# Autodesk Inventor assembly: ASY PNS-002 right module
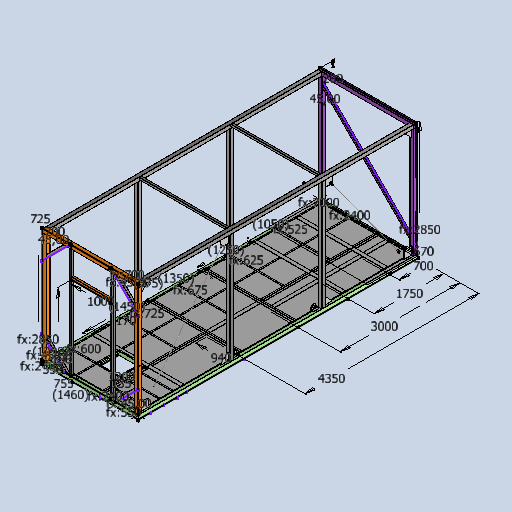
[picture p0: Inventor's stored thumbnail of the model, 512x512]
Saved by Autodesk Inventor 2025.1 (Build 291241020, 241B)
## iProperties
Created: 2025-03-25
Part Number: ASY PNS-002 right module
Document SubType Name: Assembly
Designer: user
Author: user
## Documents named in this file (15)
- C:\Users\user\YandexDisk-badmisterfox\home pc\Inventor\PNS-Panaevsk\ASY PNS-002 right module.iam
- C:\Users\user\YandexDisk-badmisterfox\home pc\Inventor\PNS-Panaevsk\ASY PNS-0210 frame right floor.iam
- C:\Users\user\YandexDisk-badmisterfox\home pc\Inventor\PNS-Panaevsk\ASY PNS-0250 frame featheredge.iam
- C:\Users\user\YandexDisk-badmisterfox\home pc\Inventor\PNS-Panaevsk\ASY PNS-0250 frame featheredge 0270.iam
- C:\Users\user\YandexDisk-badmisterfox\home pc\Inventor\PNS-Panaevsk\PNS-0261 Upper beam.ipt
- C:\Users\user\YandexDisk-badmisterfox\home pc\Inventor\PNS-Panaevsk\PNS-0262 middle pillar.ipt
- C:\Users\user\YandexDisk-badmisterfox\home pc\Inventor\PNS-Panaevsk\PNS-0262 cross beam.ipt
- C:\Users\user\YandexDisk-badmisterfox\home pc\Inventor\PNS-Panaevsk\PNS-0111 floor sheet 1.ipt
- C:\Users\user\YandexDisk-badmisterfox\home pc\Inventor\PNS-Panaevsk\PNS-071 stretch ring.ipt
- C:\Users\user\YandexDisk-badmisterfox\home pc\Inventor\PNS-Panaevsk\PNS-0310 strench.ipt
- C:\Users\user\YandexDisk-badmisterfox\home pc\Inventor\PNS-Panaevsk\PNS-0810 floor ring.ipt
- C:\Users\user\YandexDisk-badmisterfox\home pc\Inventor\PNS-Panaevsk\PNS-0812 floor ring  strengthen.ipt
- C:\Users\user\YandexDisk-badmisterfox\home pc\Inventor\PNS-Panaevsk\PNS-073 stretch tear.ipt
- C:\Users\user\YandexDisk-badmisterfox\home pc\Inventor\PNS-Panaevsk\PNS-0872 roof ring.ipt
- C:\Users\user\YandexDisk-badmisterfox\home pc\Inventor\PNS-Panaevsk\PNS-077 stretch plate.ipt
## Components (29 placed, 14 different names)
1. ASY PNS-0210 frame right floor:1 [sub-assembly] — Rigid:3, Rigid:22, Mate:38, Flush:9, Mate:42, Mate:44
2. ASY PNS-0250 frame featheredge:1 [sub-assembly] — Rigid:4, Rigid:5, Rigid:6, Rigid:7, Mate:41
3. ASY PNS-0250 frame featheredge 0270:1 [sub-assembly] — Rigid:3, Rigid:8, Rigid:9, Mate:37, Mate:40
4. PNS-0261 Upper beam:1 — Rigid:4, Mate:5, Flush:3, Mate:6, Flush:4, Mate:11, Tangent:2, Mate:22, Mate:23, Mate:26, Mate:27, Tangent:4, Mate:35, Flush:8, Mate:39, Mate:46
5. PNS-0261 Upper beam:2 — Rigid:5
6. PNS-0262 middle pillar:1 — Rigid:6, Mate:34, Mate:43
7. PNS-0262 middle pillar:2 — Rigid:7
8. PNS-0262 middle pillar:3 — Rigid:8, Mate:12, Mate:36, Mate:45
9. PNS-0262 middle pillar:4 — Rigid:9
10. PNS-0262 cross beam:1 — Mate:6, Flush:4
11. PNS-0262 cross beam:2 — Mate:5, Flush:3
12. PNS-0111 floor sheet 1:1 — Rigid:22
13. PNS-071 stretch ring:1 — Flush:12
14. PNS-071 stretch ring:2 — Flush:14
15. PNS-0310 strench:1
16. PNS-071 stretch ring:3 — Rotational:1, Mate:35, Mate:36, Flush:8, Flush:11, Flush:12
17. PNS-071 stretch ring:4 — Mate:37, Mate:38, Flush:9, Flush:10, Flush:14, Flush:15
18. PNS-0310 strench:2 — Mate:16, Tangent:3, Mate:17, Mate:21
19. PNS-0810 floor ring:2 — Mate:11, Mate:12, Tangent:2, Mate:24
20. PNS-073 stretch tear:1 — Rotational:1, Mate:16, Tangent:3, Mate:17, Flush:6, Flush:7
21. PNS-073 stretch tear:2 — Mate:21, Flush:6, Flush:7
22. PNS-0812 floor ring  strengthen:2 — Mate:22, Mate:23, Mate:24
23. PNS-0810 floor ring:3 — Mate:28, Tangent:4
24. PNS-0812 floor ring  strengthen:3 — Mate:26, Mate:27, Mate:28, Mate:34
25. PNS-0872 roof ring:1
26. PNS-077 stretch plate:1 — Mate:39, Mate:40, Flush:10
27. PNS-077 stretch plate:2 — Mate:44, Mate:45, Flush:11, Flush:13
28. PNS-077 stretch plate:3 — Mate:42, Mate:43, Flush:13
29. PNS-077 stretch plate:4 — Mate:41, Flush:15, Mate:46
## Relationships (54: Mate 28, Flush 13, WeldJoint 9, Tangent 3, RevoluteJoint 1)
- [WeldJoint]: ASY PNS-0210 frame right floor:1 ↔ ASY PNS-0250 frame featheredge:1
- Rigid:3 [WeldJoint]: ASY PNS-0210 frame right floor:1 ↔ ASY PNS-0250 frame featheredge 0270:1
- Rigid:4 [WeldJoint] (-100 mm): ASY PNS-0250 frame featheredge:1 ↔ PNS-0261 Upper beam:1
- Rigid:5 [WeldJoint] (-100 mm): ASY PNS-0250 frame featheredge:1 ↔ PNS-0261 Upper beam:2
- Rigid:6 [WeldJoint] (2200 mm): ASY PNS-0250 frame featheredge:1 ↔ PNS-0262 middle pillar:1
- Rigid:7 [WeldJoint] (2200 mm): ASY PNS-0250 frame featheredge:1 ↔ PNS-0262 middle pillar:2
- Rigid:8 [WeldJoint] (2200 mm): ASY PNS-0250 frame featheredge 0270:1 ↔ PNS-0262 middle pillar:3
- Rigid:9 [WeldJoint] (2200 mm): ASY PNS-0250 frame featheredge 0270:1 ↔ PNS-0262 middle pillar:4
- [Mate]: PNS-071 stretch ring:1 ↔ PNS-0310 strench:1
- [Flush]: PNS-071 stretch ring:1 ↔ PNS-0310 strench:1
- Rigid:22 [WeldJoint]: ASY PNS-0210 frame right floor:1 ↔ PNS-0111 floor sheet 1:1
- Mate:5: PNS-0261 Upper beam:1 ↔ PNS-0262 cross beam:2
- Flush:3: PNS-0261 Upper beam:1 ↔ PNS-0262 cross beam:2
- Mate:6: PNS-0261 Upper beam:1 ↔ PNS-0262 cross beam:1
- Flush:4: PNS-0261 Upper beam:1 ↔ PNS-0262 cross beam:1
- Mate:11 (8 mm): PNS-0261 Upper beam:1 ↔ PNS-0810 floor ring:2
- Mate:12 (20 mm): PNS-0262 middle pillar:3 ↔ PNS-0810 floor ring:2
- Tangent:2 (20 mm): PNS-0261 Upper beam:1 ↔ PNS-0810 floor ring:2
- Rotational:1 [RevoluteJoint]: PNS-071 stretch ring:3 ↔ PNS-073 stretch tear:1
- Mate:16 (-50 mm): PNS-0310 strench:2 ↔ PNS-073 stretch tear:1
- Tangent:3: PNS-0310 strench:2 ↔ PNS-073 stretch tear:1
- Mate:17: PNS-0310 strench:2 ↔ PNS-073 stretch tear:1
- Mate:21 (-50 mm): PNS-0310 strench:2 ↔ PNS-073 stretch tear:2
- Flush:6: PNS-073 stretch tear:1 ↔ PNS-073 stretch tear:2
- Flush:7: PNS-073 stretch tear:1 ↔ PNS-073 stretch tear:2
- Mate:22: PNS-0261 Upper beam:1 ↔ PNS-0812 floor ring  strengthen:2
- Mate:23: PNS-0261 Upper beam:1 ↔ PNS-0812 floor ring  strengthen:2
- Mate:24: PNS-0810 floor ring:2 ↔ PNS-0812 floor ring  strengthen:2
- [Mate]: PNS-0810 floor ring:3 ↔ PNS-0812 floor ring  strengthen:3
- Mate:26: PNS-0261 Upper beam:1 ↔ PNS-0812 floor ring  strengthen:3
- Mate:27: PNS-0261 Upper beam:1 ↔ PNS-0812 floor ring  strengthen:3
- Mate:28: PNS-0810 floor ring:3 ↔ PNS-0812 floor ring  strengthen:3
- Tangent:4 (20 mm): PNS-0261 Upper beam:1 ↔ PNS-0810 floor ring:3
- Mate:34 (20 mm): PNS-0262 middle pillar:1 ↔ PNS-0812 floor ring  strengthen:3
- Mate:35: PNS-0261 Upper beam:1 ↔ PNS-071 stretch ring:3
- Mate:36: PNS-0262 middle pillar:3 ↔ PNS-071 stretch ring:3
- Flush:8 (-50 mm): PNS-0261 Upper beam:1 ↔ PNS-071 stretch ring:3
- Mate:37: ASY PNS-0250 frame featheredge 0270:1 ↔ PNS-071 stretch ring:4
- Mate:38: ASY PNS-0210 frame right floor:1 ↔ PNS-071 stretch ring:4
- Flush:9 (50 mm): ASY PNS-0210 frame right floor:1 ↔ PNS-071 stretch ring:4
- Mate:39: PNS-0261 Upper beam:1 ↔ PNS-077 stretch plate:1
- Mate:40: ASY PNS-0250 frame featheredge 0270:1 ↔ PNS-077 stretch plate:1
- Flush:10: PNS-071 stretch ring:4 ↔ PNS-077 stretch plate:1
- Mate:41: ASY PNS-0250 frame featheredge:1 ↔ PNS-077 stretch plate:4
- Mate:42: ASY PNS-0210 frame right floor:1 ↔ PNS-077 stretch plate:3
- Mate:43: PNS-0262 middle pillar:1 ↔ PNS-077 stretch plate:3
- Mate:44: ASY PNS-0210 frame right floor:1 ↔ PNS-077 stretch plate:2
- Mate:45: PNS-0262 middle pillar:3 ↔ PNS-077 stretch plate:2
- Flush:11: PNS-071 stretch ring:3 ↔ PNS-077 stretch plate:2
- Flush:12: PNS-071 stretch ring:1 ↔ PNS-071 stretch ring:3
- Flush:13: PNS-077 stretch plate:2 ↔ PNS-077 stretch plate:3
- Flush:14: PNS-071 stretch ring:2 ↔ PNS-071 stretch ring:4
- Flush:15: PNS-071 stretch ring:4 ↔ PNS-077 stretch plate:4
- Mate:46: PNS-0261 Upper beam:1 ↔ PNS-077 stretch plate:4
## Named parameters: d18_d19 = 0 mm, d63_d62 = 0 mm
